# Autodesk Inventor assembly: fixedMount
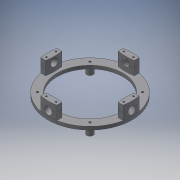
[picture p0: Inventor's stored thumbnail of the model, 180x180]
Saved by Autodesk Inventor 2016 SP1 (Build 200210100, 210)
## iProperties
Created: 2016-01-13
Part Number: fixedMount
Document SubType Name: Assembly
Designer: ddeboer
Author: ddeboer
## Documents named in this file (4)
- C:\Users\ddeboer\Desktop\leuschner-cad\fixedMount.iam
- C:\Users\ddeboer\Desktop\leuschner-cad\fixedRing.ipt
- C:\Users\ddeboer\Desktop\leuschner-cad\wedgeBlock.ipt
- C:\Users\ddeboer\Desktop\leuschner-cad\spacer.ipt
## Components (13 placed, 3 different names)
1. fixedRing:1 — Insert:4, Insert:5, Insert:6
2. spacer:1 — Insert:4
3. spacer:2
4. spacer:3
5. spacer:4
6. wedgeBlock:2 — Insert:7, Flush:1
7. wedgeBlock:1 — Insert:5, Insert:6, Insert:7, Flush:1
8. wedgeBlock:3
9. wedgeBlock:4
10. wedgeBlock:5
11. wedgeBlock:6
12. wedgeBlock:7
13. wedgeBlock:8
## Component patterns: (4 elements, first: spacer:1), (4 elements, first: wedgeBlock:2 + wedgeBlock:1)
## Relationships (5: Insert 4, Flush 1)
- Insert:4: fixedRing:1 ↔ spacer:1
- Insert:5: fixedRing:1 ↔ wedgeBlock:1
- Insert:6: fixedRing:1 ↔ wedgeBlock:1
- Insert:7 (1.5875 mm): wedgeBlock:2 ↔ wedgeBlock:1
- Flush:1: wedgeBlock:2 ↔ wedgeBlock:1
